# Autodesk Inventor assembly: Stewart-Bosy-Sym
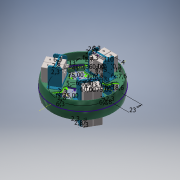
[picture p0: Inventor's stored thumbnail of the model, 180x180]
Saved by Autodesk Inventor 2018.2 (Build 222227000, 227)
## iProperties
Created: 2018-02-28
Part Number: Stewart-Bosy-Sym
Material: Generisch
Document SubType Name: Assembly
Designer: JochenAlt
Author: JochenAlt
## Documents named in this file (5)
- D:\Projects\Donna\CAD\KST DS215MG\Stewart-Body-Sym.iam
- D:\Projects\Donna\CAD\KST DS215MG\Stewart-Body-Sym.ipt
- D:\Projects\Donna\CAD\KST DS215MG\Stewart-Sym-Body-Servo-Holder-KST-DS215.ipt
- Body-Servo-Holder-KST-DS215.ipt
- D:\Projects\Donna\CAD\KST DS215MG\Servo-KST-DS215MG.ipt
## Components (19 placed, 3 different names)
1. Stewart-Plate:1 — Passend:1, Passend:2, Passend:3, Passend:4, Passend:5, Passend:6, Passend:7, Passend:8, Passend:9, Passend:10, Passend:11, Passend:12, Passend:13, Passend:14, Passend:15
2. Body-Servo-Holder-KST-DS215:1 — Passend:4, Passend:6, Passend:16, Passend:17, Passend:54, Passend:55
3. Body-Servo-Holder-KST-DS215:2 — Passend:9, Passend:11, Passend:28, Passend:29, Passend:30, Passend:37
4. Body-Servo-Holder-KST-DS215:3 — Passend:13, Passend:14, Passend:20, Passend:21, Passend:52, Passend:53
5. Body-Servo-Holder-KST-DS215:4 — Passend:8, Passend:10, Passend:18, Passend:19, Passend:68, Passend:69
6. Body-Servo-Holder-KST-DS215:5 — Passend:12, Passend:15, Passend:31, Passend:34, Passend:35, Passend:36
7. Body-Servo-Holder-KST-DS215:6 — Passend:5, Passend:7, Passend:32, Passend:33, Passend:38, Passend:39
8. Servo-KST-DS215MG:1 — Passend:16, Passend:55
9. Servo-KST-DS215MG:2 — Passend:17, Passend:54
10. Servo-KST-DS215MG:3 — Passend:20, Passend:52
11. Servo-KST-DS215MG:4 — Passend:21, Passend:53
12. Servo-KST-DS215MG:5 — Passend:19, Passend:69
13. Servo-KST-DS215MG:6 — Passend:18, Passend:68
14. Servo-KST-DS215MG:7 — Passend:28, Passend:29
15. Servo-KST-DS215MG:8 — Passend:30, Passend:37
16. Servo-KST-DS215MG:9 — Passend:32, Passend:38
17. Servo-KST-DS215MG:10 — Passend:33, Passend:39
18. Servo-KST-DS215MG:11 — Passend:34, Passend:36
19. Servo-KST-DS215MG:12 — Passend:31, Passend:35
## Relationships (39: Mate 39)
- Passend:1 [Mate]: Stewart-Plate:1
- Passend:2 [Mate]: Stewart-Plate:1
- Passend:3 [Mate]: Stewart-Plate:1
- Passend:4 [Mate]: Stewart-Plate:1 ↔ Body-Servo-Holder-KST-DS215:1
- Passend:5 [Mate]: Stewart-Plate:1 ↔ Body-Servo-Holder-KST-DS215:6
- Passend:6 [Mate]: Stewart-Plate:1 ↔ Body-Servo-Holder-KST-DS215:1
- Passend:7 [Mate]: Stewart-Plate:1 ↔ Body-Servo-Holder-KST-DS215:6
- Passend:8 [Mate]: Stewart-Plate:1 ↔ Body-Servo-Holder-KST-DS215:4
- Passend:9 [Mate]: Stewart-Plate:1 ↔ Body-Servo-Holder-KST-DS215:2
- Passend:10 [Mate]: Stewart-Plate:1 ↔ Body-Servo-Holder-KST-DS215:4
- Passend:11 [Mate]: Stewart-Plate:1 ↔ Body-Servo-Holder-KST-DS215:2
- Passend:12 [Mate]: Stewart-Plate:1 ↔ Body-Servo-Holder-KST-DS215:5
- Passend:13 [Mate]: Stewart-Plate:1 ↔ Body-Servo-Holder-KST-DS215:3
- Passend:14 [Mate]: Stewart-Plate:1 ↔ Body-Servo-Holder-KST-DS215:3
- Passend:15 [Mate]: Stewart-Plate:1 ↔ Body-Servo-Holder-KST-DS215:5
- Passend:16 [Mate]: Body-Servo-Holder-KST-DS215:1 ↔ Servo-KST-DS215MG:1
- Passend:17 [Mate]: Body-Servo-Holder-KST-DS215:1 ↔ Servo-KST-DS215MG:2
- Passend:18 [Mate]: Body-Servo-Holder-KST-DS215:4 ↔ Servo-KST-DS215MG:6
- Passend:19 [Mate]: Body-Servo-Holder-KST-DS215:4 ↔ Servo-KST-DS215MG:5
- Passend:20 [Mate]: Body-Servo-Holder-KST-DS215:3 ↔ Servo-KST-DS215MG:3
- Passend:21 [Mate]: Body-Servo-Holder-KST-DS215:3 ↔ Servo-KST-DS215MG:4
- Passend:28 [Mate]: Body-Servo-Holder-KST-DS215:2 ↔ Servo-KST-DS215MG:7
- Passend:29 [Mate]: Body-Servo-Holder-KST-DS215:2 ↔ Servo-KST-DS215MG:7
- Passend:30 [Mate]: Body-Servo-Holder-KST-DS215:2 ↔ Servo-KST-DS215MG:8
- Passend:31 [Mate]: Body-Servo-Holder-KST-DS215:5 ↔ Servo-KST-DS215MG:12
- Passend:32 [Mate]: Body-Servo-Holder-KST-DS215:6 ↔ Servo-KST-DS215MG:9
- Passend:33 [Mate]: Body-Servo-Holder-KST-DS215:6 ↔ Servo-KST-DS215MG:10
- Passend:34 [Mate]: Body-Servo-Holder-KST-DS215:5 ↔ Servo-KST-DS215MG:11
- Passend:35 [Mate]: Body-Servo-Holder-KST-DS215:5 ↔ Servo-KST-DS215MG:12
- Passend:36 [Mate]: Body-Servo-Holder-KST-DS215:5 ↔ Servo-KST-DS215MG:11
- Passend:37 [Mate]: Body-Servo-Holder-KST-DS215:2 ↔ Servo-KST-DS215MG:8
- Passend:38 [Mate]: Body-Servo-Holder-KST-DS215:6 ↔ Servo-KST-DS215MG:9
- Passend:39 [Mate]: Body-Servo-Holder-KST-DS215:6 ↔ Servo-KST-DS215MG:10
- Passend:52 [Mate]: Body-Servo-Holder-KST-DS215:3 ↔ Servo-KST-DS215MG:3
- Passend:53 [Mate]: Body-Servo-Holder-KST-DS215:3 ↔ Servo-KST-DS215MG:4
- Passend:54 [Mate]: Body-Servo-Holder-KST-DS215:1 ↔ Servo-KST-DS215MG:2
- Passend:55 [Mate]: Body-Servo-Holder-KST-DS215:1 ↔ Servo-KST-DS215MG:1
- Passend:68 [Mate]: Body-Servo-Holder-KST-DS215:4 ↔ Servo-KST-DS215MG:6
- Passend:69 [Mate]: Body-Servo-Holder-KST-DS215:4 ↔ Servo-KST-DS215MG:5
